# Autodesk Inventor assembly: Ensamblaje carcasa superior
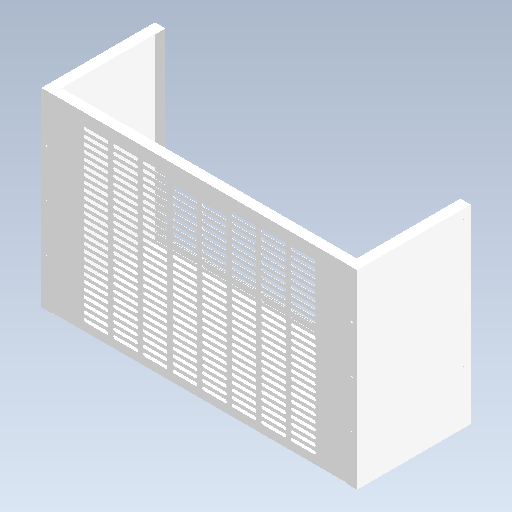
[picture p0: Inventor's stored thumbnail of the model, 512x512]
Saved by Autodesk Inventor 2021 (Build 250183000, 183)
## iProperties
Created: 2021-04-15
Part Number: Ensamblaje carcasa superior
Document SubType Name: Assembly
Designer: Admin
Author: Admin
## Documents named in this file (4)
- C:\Users\leo7s\Documents\Universidad\04 PAI\03 Proyecto\03 Github\Proyecto_PAI_2021\01 CAD\Ensamblaje carcasa superior.iam
- C:\Users\leo7s\Documents\Universidad\04 PAI\03 Proyecto\03 Github\Proyecto_PAI_2021\01 CAD\Tapa_superior_superior.ipt
- C:\Users\leo7s\Documents\Universidad\04 PAI\03 Proyecto\03 Github\Proyecto_PAI_2021\01 CAD\Tapa_superior_izquierda.ipt
- C:\Users\leo7s\Documents\Universidad\04 PAI\03 Proyecto\03 Github\Proyecto_PAI_2021\01 CAD\Tapa_superior_derecha.ipt
## Components (3 placed, 3 different names)
1. Tapa_superior_superior:1 — Coincidencia:1, Coincidencia:2, Coincidencia:3, Coincidencia:4, Coincidencia:5, Coincidencia:6
2. Tapa_superior_izquierda:1 — Coincidencia:1, Coincidencia:2, Coincidencia:3
3. Tapa_superior_derecha:1 — Coincidencia:4, Coincidencia:5, Coincidencia:6
## Relationships (6: Mate 6)
- Coincidencia:1 [Mate]: Tapa_superior_superior:1 ↔ Tapa_superior_izquierda:1
- Coincidencia:2 [Mate]: Tapa_superior_superior:1 ↔ Tapa_superior_izquierda:1
- Coincidencia:3 [Mate]: Tapa_superior_superior:1 ↔ Tapa_superior_izquierda:1
- Coincidencia:4 [Mate]: Tapa_superior_superior:1 ↔ Tapa_superior_derecha:1
- Coincidencia:5 [Mate]: Tapa_superior_superior:1 ↔ Tapa_superior_derecha:1
- Coincidencia:6 [Mate]: Tapa_superior_superior:1 ↔ Tapa_superior_derecha:1
